# Autodesk Inventor assembly: CompleteRobotAssembly_NERDS
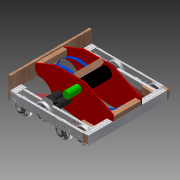
[picture p0: Inventor's stored thumbnail of the model, 180x180]
Saved by Autodesk Inventor 2014 (Build 180170000, 170)
## iProperties
Created: 2016-01-30
Part Number: CompleteRobotAssembly_NERDS
Document SubType Name: Assembly
Designer: bermudezr
Author: bermudezr
## Documents named in this file (5)
- C:\Users\choices.CTE\Documents\Nerds_1726\Models\2015-2016\Assemblies\Robot\Complete.iam
- C:\Users\choices.CTE\Documents\Nerds_1726\Models\2015-2016\Assemblies\Robot\Shooter.iam
- C:\Users\choices.CTE\Documents\Nerds_1726\Models\2015-2016\Assemblies\Robot\Chassis.iam
- C:\Users\choices.CTE\Documents\Nerds_1726\Models\2015-2016\Parts\Robot\Shooter\BallGuidePly.ipt
- C:\Users\choices.CTE\Documents\Nerds_1726\Models\2015-2016\Parts\Robot\Shooter\BallGuidePlyRight.ipt
## Components (4 placed, 4 different names)
1. Shooter:1 [sub-assembly] — Mate:4, Mate:5, Flush:2, Mate:6, Flush:3
2. Chassis:1 [sub-assembly] — Mate:4, Mate:5, Flush:2, Mate:6, Flush:3, Insert:1, Insert:2, Insert:3, Insert:4
3. BallGuidePly:1 — Insert:1, Insert:2
4. BallGuidePlyRight:1 — Insert:3, Insert:4
## Relationships (9: Insert 4, Mate 3, Flush 2)
- Mate:4: Shooter:1 ↔ Chassis:1
- Mate:5: Shooter:1 ↔ Chassis:1
- Flush:2: Shooter:1 ↔ Chassis:1
- Mate:6: Shooter:1 ↔ Chassis:1
- Flush:3: Shooter:1 ↔ Chassis:1
- Insert:1: Chassis:1 ↔ BallGuidePly:1
- Insert:2: Chassis:1 ↔ BallGuidePly:1
- Insert:3: Chassis:1 ↔ BallGuidePlyRight:1
- Insert:4: Chassis:1 ↔ BallGuidePlyRight:1
